# Autodesk Inventor assembly: Frame 1759007616013
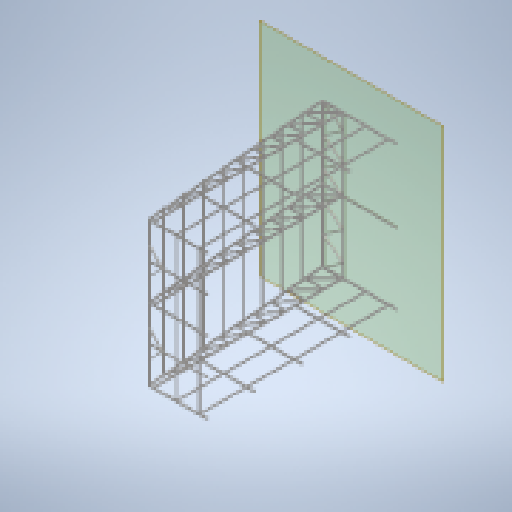
[picture p0: Inventor's stored thumbnail of the model, 512x512]
Saved by Autodesk Inventor 2025.2 (Build 292293000, 293)
## iProperties
_FrameDoc: Frame Assembly
_Version: 25.0.0
Created: 2025-09-27
Part Number: Frame 1759007616013
Document SubType Name: Assembly
Designer: MB
Mass: 340261 g
Surface Area: 285865 cm^2
Volume: 43345.4 cm^3
Density: 7.85 g/cm^3
Author: MB
## Documents named in this file (70)
- C:\Users\MB\Documents\GitHub\hegesztes\Garage_roof_side\Frame\Frame 1759007616013.iam
- C:\Users\MB\Documents\GitHub\hegesztes\Garage_roof_side\Frame\Skeleton 1759007616014.ipt
- C:\Users\MB\Documents\GitHub\hegesztes\Garage_roof_side\Frame\ISO 10799-2 60x60x4 1759007627317.ipt
- C:\Users\MB\Documents\GitHub\hegesztes\Garage_roof_side\Frame\ISO 10799-2 60x60x4 1759007627345.ipt
- C:\Users\MB\Documents\GitHub\hegesztes\Garage_roof_side\Frame\ISO 10799-2 60x60x4 1759007627374.ipt
- C:\Users\MB\Documents\GitHub\hegesztes\Garage_roof_side\Frame\ISO 10799-2 60x60x4 1759007627404.ipt
- C:\Users\MB\Documents\GitHub\hegesztes\Garage_roof_side\Frame\ISO 10799-2 60x60x4 1759007627431.ipt
- C:\Users\MB\Documents\GitHub\hegesztes\Garage_roof_side\Frame\ISO 10799-2 60x60x4 1759007627458.ipt
- C:\Users\MB\Documents\GitHub\hegesztes\Garage_roof_side\Frame\ISO 10799-2 60x60x4 1759007627486.ipt
- C:\Users\MB\Documents\GitHub\hegesztes\Garage_roof_side\Frame\ISO 10799-2 60x40x2 1759007728132.ipt
- C:\Users\MB\Documents\GitHub\hegesztes\Garage_roof_side\Frame\ISO 10799-2 60x40x2 1759007728164.ipt
- C:\Users\MB\Documents\GitHub\hegesztes\Garage_roof_side\Frame\ISO 10799-2 60x40x2 1759007728198.ipt
- C:\Users\MB\Documents\GitHub\hegesztes\Garage_roof_side\Frame\ISO 10799-2 60x40x2 1759007728265.ipt
- C:\Users\MB\Documents\GitHub\hegesztes\Garage_roof_side\Frame\ISO 10799-2 60x40x2 1759007728334.ipt
- C:\Users\MB\Documents\GitHub\hegesztes\Garage_roof_side\Frame\ISO 10799-2 60x40x2 1759007728369.ipt
- C:\Users\MB\Documents\GitHub\hegesztes\Garage_roof_side\Frame\ISO 10799-2 60x40x2 1759007728437.ipt
- C:\Users\MB\Documents\GitHub\hegesztes\Garage_roof_side\Frame\ISO 10799-2 60x40x2 1759007728471.ipt
- C:\Users\MB\Documents\GitHub\hegesztes\Garage_roof_side\Frame\ISO 10799-2 60x40x2 1759007728540.ipt
- C:\Users\MB\Documents\GitHub\hegesztes\Garage_roof_side\Frame\ISO 10799-2 60x40x2 1759007728574.ipt
- C:\Users\MB\Documents\GitHub\hegesztes\Garage_roof_side\Frame\ISO 10799-2 60x40x2 1759007728609.ipt
- C:\Users\MB\Documents\GitHub\hegesztes\Garage_roof_side\Frame\ISO 10799-2 60x40x2 1759007728645.ipt
- C:\Users\MB\Documents\GitHub\hegesztes\Garage_roof_side\Frame\ISO 10799-2 60x40x2 1759007728679.ipt
- C:\Users\MB\Documents\GitHub\hegesztes\Garage_roof_side\Frame\ISO 10799-2 60x40x2 1759007728712.ipt
- C:\Users\MB\Documents\GitHub\hegesztes\Garage_roof_side\Frame\ISO 10799-2 60x40x2 1759007728748.ipt
- C:\Users\MB\Documents\GitHub\hegesztes\Garage_roof_side\Frame\ISO 10799-2 60x40x2 1759007728783.ipt
- C:\Users\MB\Documents\GitHub\hegesztes\Garage_roof_side\Frame\ISO 10799-2 60x40x2 1759007728818.ipt
- C:\Users\MB\Documents\GitHub\hegesztes\Garage_roof_side\Frame\ISO 10799-2 60x40x2 1759007728853.ipt
- C:\Users\MB\Documents\GitHub\hegesztes\Garage_roof_side\Frame\ISO 10799-2 60x40x2 1759007728922.ipt
- C:\Users\MB\Documents\GitHub\hegesztes\Garage_roof_side\Frame\ISO 10799-2 60x40x2 1759007728956.ipt
- C:\Users\MB\Documents\GitHub\hegesztes\Garage_roof_side\Frame\ISO 10799-2 60x60x4 1759085561171.ipt
- C:\Users\MB\Documents\GitHub\hegesztes\Garage_roof_side\Frame\ISO 10799-2 60x60x4 1759085561199.ipt
- C:\Users\MB\Documents\GitHub\hegesztes\Garage_roof_side\Frame\ISO 10799-2 60x40x2 1759085612504.ipt
- C:\Users\MB\Documents\GitHub\hegesztes\Garage_roof_side\Frame\ISO 10799-2 60x40x2 1759085612535.ipt
- C:\Users\MB\Documents\GitHub\hegesztes\Garage_roof_side\Frame\ISO 10799-2 60x40x2 1759085612567.ipt
- C:\Users\MB\Documents\GitHub\hegesztes\Garage_roof_side\Frame\ISO 10799-2 60x40x2 1759085612603.ipt
- C:\Users\MB\Documents\GitHub\hegesztes\Garage_roof_side\Frame\ISO 10799-2 60x40x2 1759085612635.ipt
- C:\Users\MB\Documents\GitHub\hegesztes\Garage_roof_side\Frame\ISO 10799-2 60x40x2 1759085612667.ipt
- C:\Users\MB\Documents\GitHub\hegesztes\Garage_roof_side\Frame\ISO 10799-2 60x40x2 1759085612698.ipt
- C:\Users\MB\Documents\GitHub\hegesztes\Garage_roof_side\Frame\ISO 10799-2 60x40x2 1759085612730.ipt
- C:\Users\MB\Documents\GitHub\hegesztes\Garage_roof_side\Frame\ISO 10799-2 60x40x2 1759085612763.ipt
- C:\Users\MB\Documents\GitHub\hegesztes\Garage_roof_side\Frame\ISO 10799-2 60x40x2 1759085612796.ipt
- C:\Users\MB\Documents\GitHub\hegesztes\Garage_roof_side\Frame\ISO 10799-2 60x40x2 1759085612828.ipt
- C:\Users\MB\Documents\GitHub\hegesztes\Garage_roof_side\Frame\ISO 10799-2 60x40x2 1759085612861.ipt
- C:\Users\MB\Documents\GitHub\hegesztes\Garage_roof_side\Frame\ISO 10799-2 60x60x4 1759086288725.ipt
- C:\Users\MB\Documents\GitHub\hegesztes\Garage_roof_side\Frame\ISO 10799-2 60x60x4 1759086710382.ipt
- C:\Users\MB\Documents\GitHub\hegesztes\Garage_roof_side\Frame\ISO 10799-2 60x60x4 1759087486059.ipt
- C:\Users\MB\Documents\GitHub\hegesztes\Garage_roof_side\Frame\ISO 10799-2 60x40x2 1759089859357.ipt
- C:\Users\MB\Documents\GitHub\hegesztes\Garage_roof_side\Frame\ISO 10799-2 60x40x2 1759089859400.ipt
- C:\Users\MB\Documents\GitHub\hegesztes\Garage_roof_side\Frame\ISO 10799-2 60x40x2 1759089859434.ipt
- C:\Users\MB\Documents\GitHub\hegesztes\Garage_roof_side\Frame\ISO 10799-2 60x40x2 1759089859466.ipt
- C:\Users\MB\Documents\GitHub\hegesztes\Garage_roof_side\Frame\ISO 10799-2 60x40x2 1759089859503.ipt
- C:\Users\MB\Documents\GitHub\hegesztes\Garage_roof_side\Frame\ISO 10799-2 60x40x2 1759089859540.ipt
- C:\Users\MB\Documents\GitHub\hegesztes\Garage_roof_side\Frame\ISO 10799-2 60x40x2 1759089859577.ipt
- C:\Users\MB\Documents\GitHub\hegesztes\Garage_roof_side\Frame\ISO 10799-2 60x40x2 1759089859609.ipt
- C:\Users\MB\Documents\GitHub\hegesztes\Garage_roof_side\Frame\ISO 10799-2 60x40x2 1759089859643.ipt
- C:\Users\MB\Documents\GitHub\hegesztes\Garage_roof_side\Frame\ISO 10799-2 60x40x2 1759089859677.ipt
- C:\Users\MB\Documents\GitHub\hegesztes\Garage_roof_side\Frame\ISO 10799-2 60x40x2 1759089859710.ipt
- C:\Users\MB\Documents\GitHub\hegesztes\Garage_roof_side\Frame\ISO 10799-2 60x40x2 1759089859742.ipt
- C:\Users\MB\Documents\GitHub\hegesztes\Garage_roof_side\Frame\ISO 10799-2 60x40x2 1759089859775.ipt
- C:\Users\MB\Documents\GitHub\hegesztes\Garage_roof_side\Frame\ISO 10799-2 60x40x2 1759089859808.ipt
- C:\Users\MB\Documents\GitHub\hegesztes\Garage_roof_side\Frame\ISO 10799-2 60x40x2 1759089859843.ipt
- C:\Users\MB\Documents\GitHub\hegesztes\Garage_roof_side\Frame\ISO 10799-2 60x40x2 1759089859875.ipt
- C:\Users\MB\Documents\GitHub\hegesztes\Garage_roof_side\Frame\ISO 10799-2 60x40x2 1759091012818.ipt
- C:\Users\MB\Documents\GitHub\hegesztes\Garage_roof_side\Frame\ISO 10799-2 60x40x2 1759091012850.ipt
- C:\Users\MB\Documents\GitHub\hegesztes\Garage_roof_side\Frame\ISO 10799-2 60x40x2 1759091012883.ipt
- C:\Users\MB\Documents\GitHub\hegesztes\Garage_roof_side\Frame\ISO 10799-2 60x40x2 1759091012925.ipt
- C:\Users\MB\Documents\GitHub\hegesztes\Garage_roof_side\Frame\ISO 10799-2 60x40x2 1759091012957.ipt
- C:\Users\MB\Documents\GitHub\hegesztes\Garage_roof_side\Frame\ISO 10799-2 60x40x2 1759091012990.ipt
- C:\Users\MB\Documents\GitHub\hegesztes\Garage_roof_side\Frame\ISO 10799-2 60x40x2 1759091013024.ipt
- C:\Users\MB\Documents\GitHub\hegesztes\Garage_roof_side\Frame\ISO 10799-2 60x40x2 1759091013058.ipt
## Components (127 placed, 38 different names)
1. Reference Skeleton
2. ISO 10799-2 60x60x4 - 5350:1
3. ISO 10799-2 60x60x4 - 5350:2
4. ISO 10799-2 60x40x2 - 720:2
5. ISO 10799-2 60x40x2 - 873,65:1
6. ISO 10799-2 60x40x2 - 873,65:2
7. ISO 10799-2 60x40x2 - 873,65:3
8. ISO 10799-2 60x40x2 - 873,65:4
9. ISO 10799-2 60x40x2 - 873,65:5
10. ISO 10799-2 60x40x2 - 873,65:6
11. ISO 10799-2 60x40x2 - 873,65:7
12. ISO 10799-2 60x40x2 - 873,65:8
13. ISO 10799-2 60x40x2 - 873,65:9
14. ISO 10799-2 60x40x2 - 861,33:10
15. ISO 10799-2 60x40x2 - 750:3
16. ISO 10799-2 60x60x4 - 2000:7
17. ISO 10799-2 60x40x2 - 2606:1
18. ISO 10799-2 60x40x2 - 2606:2
19. ISO 10799-2 60x40x2 - 2150:1
20. ISO 10799-2 60x40x2 - 2150:2
21. ISO 10799-2 60x40x2 - 1303:1
22. ISO 10799-2 60x40x2 - 1303:2
23. ISO 10799-2 60x40x2 - 1303:3
24. ISO 10799-2 60x40x2 - 1303:4
25. ISO 10799-2 60x40x2 - 1303:5
26. ISO 10799-2 60x40x2 - 1303:6
27. ISO 10799-2 60x40x2 - 1325:1
28. ISO 10799-2 60x40x2 - 1325:2
29. ISO 10799-2 60x40x2 - 700:1
30. ISO 10799-2 60x40x2 - 700:2
31. ISO 10799-2 60x40x2 - 700:3
32. ISO 10799-2 60x40x2 - 700:4
33. ISO 10799-2 60x40x2 - 5344:1
34. ISO 10799-2 60x40x2 - 5344:2
35. ISO 10799-2 60x40x2 - 5344:3
36. ISO 10799-2 60x40x2 - 5344:4
37. ISO 10799-2 60x40x2 - 5344:5
38. ISO 10799-2 60x40x2 - 5344:6
39. ISO 10799-2 60x40x2 - 5344:7
40. ISO 10799-2 60x40x2 - 5344:8
41. ISO 10799-2 60x60x4 - 7032,15:1
42. ISO 10799-2 60x60x4 - 182,68:1
43. ISO 10799-2 60x40x2 - 6940:1
44. ISO 10799-2 60x60x4 - 7000:1
45. ISO 10799-2 60x40x2 - 155,28:1
46. ISO 10799-2 60x40x2 - 215,28:1
47. ISO 10799-2 60x40x2 - 659,54:1
48. ISO 10799-2 60x40x2 - 275,28:1
49. ISO 10799-2 60x40x2 - 689,4:1
50. ISO 10799-2 60x40x2 - 335,28:1
51. ISO 10799-2 60x40x2 - 719,18:1
52. ISO 10799-2 60x40x2 - 395,28:1
53. ISO 10799-2 60x40x2 - 750,44:1
54. ISO 10799-2 60x40x2 - 455,28:1
55. ISO 10799-2 60x40x2 - 783,75:1
56. ISO 10799-2 60x40x2 - 515,28:1
57. ISO 10799-2 60x40x2 - 819,25:1
58. ISO 10799-2 60x60x4 - 1970:5
59. ISO 10799-2 60x60x4 - 1970:4
60. ISO 10799-2 60x60x4 - 1970:3
61. ISO 10799-2 60x60x4 - 2000:1
62. ISO 10799-2 60x40x2 - 7000:2
63. ISO 10799-2 60x40x2 - 856,89:1
64. ISO 10799-2 60x40x2 - 575,28:1
65. ISO 10799-2 60x40x2 - 896,54:1
66. ISO 10799-2 60x40x2 - 635,28:1
67. ISO 10799-2 60x40x2 - 938,04:1
68. ISO 10799-2 60x60x4 - 695,81:1
69. ISO 10799-2 60x60x4 - 1970:2
70. ISO 10799-2 60x60x4 - 7032,15:2
71. ISO 10799-2 60x60x4 - 182,68:2
72. ISO 10799-2 60x40x2 - 6940:2
73. ISO 10799-2 60x60x4 - 7000:2
74. ISO 10799-2 60x40x2 - 155,28:2
75. ISO 10799-2 60x40x2 - 215,28:2
76. ISO 10799-2 60x40x2 - 659,54:2
77. ISO 10799-2 60x40x2 - 275,28:2
78. ISO 10799-2 60x40x2 - 689,4:2
79. ISO 10799-2 60x40x2 - 335,28:2
80. ISO 10799-2 60x40x2 - 719,18:2
81. ISO 10799-2 60x40x2 - 395,28:2
82. ISO 10799-2 60x40x2 - 750,44:2
83. ISO 10799-2 60x40x2 - 455,28:2
84. ISO 10799-2 60x40x2 - 783,75:2
85. ISO 10799-2 60x40x2 - 515,28:2
86. ISO 10799-2 60x40x2 - 819,25:2
87. ISO 10799-2 60x60x4 - 1970:6
88. ISO 10799-2 60x60x4 - 1970:7
89. ISO 10799-2 60x60x4 - 1970:8
90. ISO 10799-2 60x60x4 - 2000:6
91. ISO 10799-2 60x40x2 - 7000:3
92. ISO 10799-2 60x40x2 - 856,89:2
93. ISO 10799-2 60x40x2 - 575,28:2
94. ISO 10799-2 60x40x2 - 896,54:2
95. ISO 10799-2 60x40x2 - 635,28:2
96. ISO 10799-2 60x40x2 - 938,04:2
97. ISO 10799-2 60x60x4 - 695,81:2
98. ISO 10799-2 60x60x4 - 1970:9
99. ISO 10799-2 60x60x4 - 7032,15:3
100. ISO 10799-2 60x60x4 - 182,68:3
101. ISO 10799-2 60x40x2 - 6940:3
102. ISO 10799-2 60x60x4 - 7000:3
103. ISO 10799-2 60x40x2 - 155,28:3
104. ISO 10799-2 60x40x2 - 215,28:3
105. ISO 10799-2 60x40x2 - 659,54:3
106. ISO 10799-2 60x40x2 - 275,28:3
107. ISO 10799-2 60x40x2 - 689,4:3
108. ISO 10799-2 60x40x2 - 335,28:3
109. ISO 10799-2 60x40x2 - 719,18:3
110. ISO 10799-2 60x40x2 - 395,28:3
111. ISO 10799-2 60x40x2 - 750,44:3
112. ISO 10799-2 60x40x2 - 455,28:3
113. ISO 10799-2 60x40x2 - 783,75:3
114. ISO 10799-2 60x40x2 - 515,28:3
115. ISO 10799-2 60x40x2 - 819,25:3
116. ISO 10799-2 60x60x4 - 1970:10
117. ISO 10799-2 60x60x4 - 1970:11
118. ISO 10799-2 60x60x4 - 1970:12
119. ISO 10799-2 60x60x4 - 2000:8
120. ISO 10799-2 60x40x2 - 7000:4
121. ISO 10799-2 60x40x2 - 856,89:3
122. ISO 10799-2 60x40x2 - 575,28:3
123. ISO 10799-2 60x40x2 - 896,54:3
124. ISO 10799-2 60x40x2 - 635,28:3
125. ISO 10799-2 60x40x2 - 938,04:3
126. ISO 10799-2 60x60x4 - 695,81:3
127. ISO 10799-2 60x60x4 - 1970:13
## Component patterns: (3 elements, first: ISO 10799-2 60x60x4 - 7032,15:1 + ISO 10799-2 60x60x4 - 182,68:1 + ISO 10799-2 60x40x2 - 6940:1 + ISO 10799-2 60x60x4 - 7000:1 + ISO 10799-2 60x40x2 - 155,28:1 + ISO 10799-2 60x40x2 - 215,28:1 + ISO 10799-2 60x40x2 - 659,54:1 + ISO 10799-2 60x40x2 - 275,28:1 + ISO 10799-2 60x40x2 - 689,4:1 + ISO 10799-2 60x40x2 - 335,28:1 + ISO 10799-2 60x40x2 - 719,18:1 + ISO 10799-2 60x40x2 - 395,28:1 + ISO 10799-2 60x40x2 - 750,44:1 + ISO 10799-2 60x40x2 - 455,28:1 + ISO 10799-2 60x40x2 - 783,75:1 + ISO 10799-2 60x40x2 - 515,28:1 + ISO 10799-2 60x40x2 - 819,25:1 + ISO 10799-2 60x60x4 - 1970:5 + ISO 10799-2 60x60x4 - 1970:4 + ISO 10799-2 60x60x4 - 1970:3 + ISO 10799-2 60x60x4 - 2000:1 + ISO 10799-2 60x40x2 - 7000:2 + ISO 10799-2 60x40x2 - 856,89:1 + ISO 10799-2 60x40x2 - 575,28:1 + ISO 10799-2 60x40x2 - 896,54:1 + ISO 10799-2 60x40x2 - 635,28:1 + ISO 10799-2 60x40x2 - 938,04:1 + ISO 10799-2 60x60x4 - 695,81:1 + ISO 10799-2 60x60x4 - 1970:2)
